# Autodesk Inventor assembly: Vex Traction Wheel 6x1
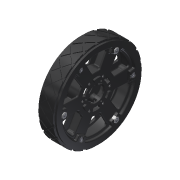
[picture p0: Inventor's stored thumbnail of the model, 180x180]
Saved by Autodesk Inventor 2013 (Build 170138000, 138)
## iProperties
Created: 2012-12-09
Part Number: Vex Traction Wheel 6x1
Document SubType Name: Assembly
Designer: Nemo
Author: Nemo
## Documents named in this file (6)
- H:\Nemo\Documents\Robotics\VexPro\Traction Wheel\Vex Traction Wheel 6x1.iam
- H:\Nemo\Documents\Robotics\VexPro\Traction Wheel\Components\Traction Tire Body 6in.ipt
- H:\Nemo\Documents\Robotics\VexPro\Fasteners\Hex Standoff 8-32 x750.ipt
- H:\Nemo\Documents\Robotics\VexPro\Fasteners\8-32 locknut.ipt
- H:\Nemo\Documents\Robotics\VexPro\Fasteners\8-32 x1250 button head.ipt
- H:\Nemo\Documents\Robotics\VexPro\Traction Wheel\Components\6 Traction Tire - 1 Wide.ipt
## Components (21 placed, 5 different names)
1. Traction Tire Body 6in:1 — Mate:1, Flush:1, Mate:2, Angle:1, Insert:1, Insert:2, Angle:2, Insert:3, Mate:5
2. Traction Tire Body 6in:2 — Mate:3, Mate:4, Mate:5, Insert:4, Angle:3, Insert:5
3. 6 Traction Tire - 1 Wide:1 — Mate:6, Mate:7, Mate:8
4. Hex Standoff 8-32 x750:1 — Angle:1, Insert:1
5. Hex Standoff 8-32 x750:2
6. Hex Standoff 8-32 x750:3
7. Hex Standoff 8-32 x750:4
8. Hex Standoff 8-32 x750:5
9. Hex Standoff 8-32 x750:6
10. 8-32 x1250 button head:2 — Insert:4
11. 8-32 locknut:2 — Angle:3, Insert:5
12. 8-32 x1250 button head:1 — Insert:3
13. 8-32 locknut:1 — Insert:2, Angle:2
14. 8-32 x1250 button head:3
15. 8-32 locknut:3
16. 8-32 x1250 button head:4
17. 8-32 locknut:4
18. 8-32 x1250 button head:5
19. 8-32 locknut:5
20. 8-32 x1250 button head:6
21. 8-32 locknut:6
## Component patterns: (6 elements, first: Hex Standoff 8-32 x750:1), (3 elements, first: 8-32 x1250 button head:2 + 8-32 locknut:2 + 8-32 x1250 button head:1 + 8-32 locknut:1)
## Relationships (17: Mate 8, Insert 5, Angle 3, Flush 1)
- Mate:1: Traction Tire Body 6in:1
- Flush:1: Traction Tire Body 6in:1
- Mate:2: Traction Tire Body 6in:1
- Angle:1 (0 deg): Traction Tire Body 6in:1 ↔ Hex Standoff 8-32 x750:1
- Insert:1: Traction Tire Body 6in:1 ↔ Hex Standoff 8-32 x750:1
- Insert:2: Traction Tire Body 6in:1 ↔ 8-32 locknut:1
- Angle:2 (0 deg): Traction Tire Body 6in:1 ↔ 8-32 locknut:1
- Insert:3: Traction Tire Body 6in:1 ↔ 8-32 x1250 button head:1
- Mate:3: Traction Tire Body 6in:2
- Mate:4: Traction Tire Body 6in:2
- Mate:5: Traction Tire Body 6in:1 ↔ Traction Tire Body 6in:2
- Insert:4: Traction Tire Body 6in:2 ↔ 8-32 x1250 button head:2
- Angle:3 (0 deg): Traction Tire Body 6in:2 ↔ 8-32 locknut:2
- Insert:5: Traction Tire Body 6in:2 ↔ 8-32 locknut:2
- Mate:6: 6 Traction Tire - 1 Wide:1
- Mate:7: 6 Traction Tire - 1 Wide:1
- Mate:8: 6 Traction Tire - 1 Wide:1
